# Autodesk Inventor assembly: TablaDejar
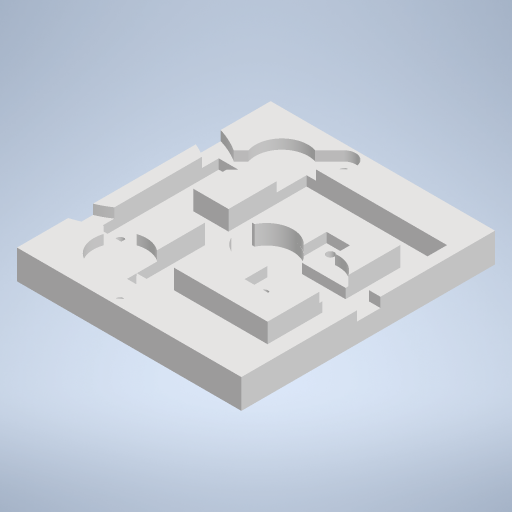
[picture p0: Inventor's stored thumbnail of the model, 512x512]
Saved by Autodesk Inventor 2023 (Build 270158000, 158)
## iProperties
Created: 2022-11-06
Part Number: TablaDejar
Document SubType Name: Assembly
Designer: allan
Author: allan
## Documents named in this file (4)
- D:\Documents\UNAL\semestre 8\Robotica\Proyecto\TablaDejar.iam
- D:\Documents\UNAL\semestre 8\Robotica\Proyecto\Etapa2Base.ipt
- D:\Documents\UNAL\semestre 8\Robotica\Proyecto\TablaBase.ipt
- D:\Documents\UNAL\semestre 8\Robotica\Proyecto\ParteFinalMesaEnsamble.ipt
## Components (3 placed, 3 different names)
1. Etapa2Base:1 — Mate:1, Mate:2, Flush:1, Flush:2, Flush:3, Flush:4
2. TablaBase:1 — Mate:1, Flush:1, Flush:2
3. ParteFinalMesaEnsamble:1 — Mate:2, Flush:3, Flush:4
## Relationships (6: Flush 4, Mate 2)
- Mate:1: Etapa2Base:1 ↔ TablaBase:1
- Mate:2: Etapa2Base:1 ↔ ParteFinalMesaEnsamble:1
- Flush:1: Etapa2Base:1 ↔ TablaBase:1
- Flush:2: Etapa2Base:1 ↔ TablaBase:1
- Flush:3: Etapa2Base:1 ↔ ParteFinalMesaEnsamble:1
- Flush:4: Etapa2Base:1 ↔ ParteFinalMesaEnsamble:1
